# Autodesk Inventor assembly: PI5_Case
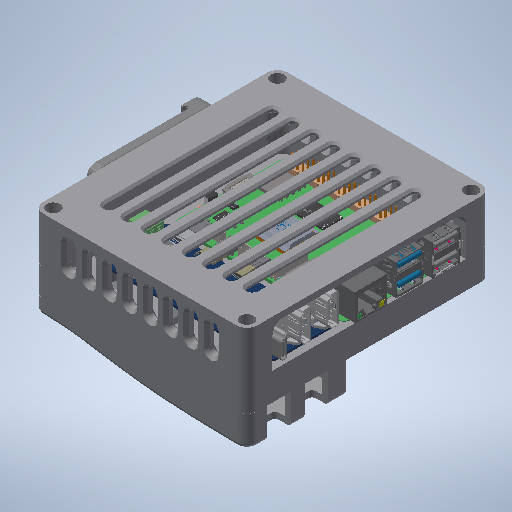
[picture p0: Inventor's stored thumbnail of the model, 512x512]
Saved by Autodesk Inventor 2025.4 (Build 294407000, 407)
## iProperties
Created: 2026-08-04
Part Number: PI5_Case
Document SubType Name: Assembly
Designer: louis
Author: louis
## Documents named in this file (7)
- C:\Users\louis\OneDrive\Desktop\R_Trident\02_CAD\04_Subassemblies\PI5_Case.iam
- C:\Users\louis\OneDrive\Desktop\R_Trident\02_CAD\03_Parts_Custom\PI5_Case\Pi5SupportBasePlate.ipt
- C:\Users\louis\OneDrive\Desktop\R_Trident\02_CAD\01_Standard_Parts\04_ELE_Electrical_Automation\Pi5\Pi5-Connector-Adapter.ipt
- C:\Users\louis\OneDrive\Desktop\R_Trident\02_CAD\01_Standard_Parts\04_ELE_Electrical_Automation\Pi5\RASPBERRY_PI_5_1.ipt
- C:\Users\louis\OneDrive\Desktop\R_Trident\02_CAD\03_Parts_Custom\PI5_Case\Pi5TopCover.ipt
- C:\Users\louis\OneDrive\Desktop\R_Trident\02_CAD\03_Parts_Custom\PI5_Case\Pi5PowerCover.ipt
- C:\Users\louis\OneDrive\Desktop\R_Trident\02_CAD\01_Standard_Parts\04_ELE_Electrical_Automation\Pi5\din_clip_heat_insert.ipt
## Components (7 placed, 6 different names)
1. Pi5SupportBasePlate:1 — Flush:1, Flush:2, Flush:3, Mate:1, Mate:2, Mate:3, Mate:4, Mate:5, Mate:6, Mate:7, Mate:8, Mate:9, Mate:12, Mate:13
2. Pi5-Connector-Adapter:1 — Mate:3, Mate:4
3. RASPBERRY_PI_5_1:1 — Mate:1, Mate:2
4. Pi5TopCover:1 — Mate:5, Mate:6, Mate:10, Mate:11
5. Pi5PowerCover:1 — Mate:7, Mate:8, Mate:9
6. din_clip_heat_insert:1 — Mate:10, Mate:11
7. din_clip_heat_insert:2 — Mate:12, Mate:13
## Relationships (16: Mate 13, Flush 3)
- Flush:1: Pi5SupportBasePlate:1
- Flush:2: Pi5SupportBasePlate:1
- Flush:3: Pi5SupportBasePlate:1
- Mate:1: Pi5SupportBasePlate:1 ↔ RASPBERRY_PI_5_1:1
- Mate:2: Pi5SupportBasePlate:1 ↔ RASPBERRY_PI_5_1:1
- Mate:3: Pi5SupportBasePlate:1 ↔ Pi5-Connector-Adapter:1
- Mate:4: Pi5SupportBasePlate:1 ↔ Pi5-Connector-Adapter:1
- Mate:5: Pi5SupportBasePlate:1 ↔ Pi5TopCover:1
- Mate:6: Pi5SupportBasePlate:1 ↔ Pi5TopCover:1
- Mate:7: Pi5SupportBasePlate:1 ↔ Pi5PowerCover:1
- Mate:8: Pi5SupportBasePlate:1 ↔ Pi5PowerCover:1
- Mate:9: Pi5SupportBasePlate:1 ↔ Pi5PowerCover:1
- Mate:10: Pi5TopCover:1 ↔ din_clip_heat_insert:1
- Mate:11: Pi5TopCover:1 ↔ din_clip_heat_insert:1
- Mate:12: Pi5SupportBasePlate:1 ↔ din_clip_heat_insert:2
- Mate:13: Pi5SupportBasePlate:1 ↔ din_clip_heat_insert:2
